# Autodesk Inventor assembly: Assembly2
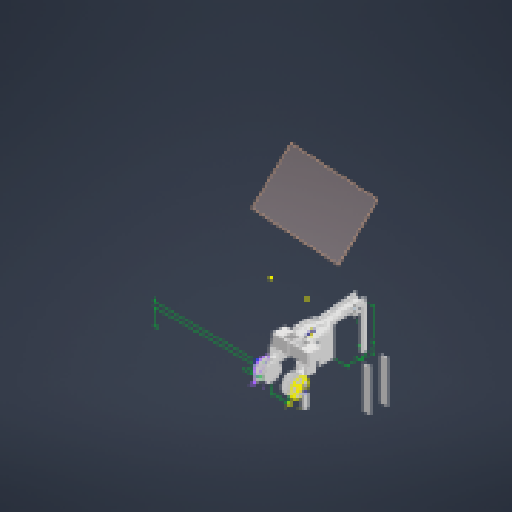
[picture p0: Inventor's stored thumbnail of the model, 512x512]
Saved by Autodesk Inventor 2026.2 (Build 302298000, 298)
## iProperties
Created: 2026-02-23
Part Number: Assembly2
Document SubType Name: Assembly
Designer: danda
Author: danda
## Documents named in this file (17)
- C:\Users\danda\BOM-project\Project\CAD\sorting\Assembly2.iam
- C:\Users\danda\BOM-project\Project\CAD\sorting\Towerpro Micro Servo 9g\Towerpro Micro Servo 9g\Towerpro Micro Servo 9g.ipt
- C:\Users\danda\BOM-project\Project\CAD\sorting\gate2.ipt
- C:\Users\danda\BOM-project\Project\CAD\sorting\wheel.ipt
- C:\Users\danda\BOM-project\Project\CAD\sorting\motorwheelstand.ipt
- C:\Users\danda\BOM-project\Project\CAD\sorting\leftcollection.ipt
- C:\Users\danda\BOM-project\Project\CAD\sorting\rightcollection.ipt
- C:\Users\danda\Downloads\ir-sensor-7.snapshot.2\Assembly2.iam
- C:\Users\danda\BOM-project\Project\CAD\sorting\wheel_MIR.ipt
- C:\Users\danda\BOM-project\Project\CAD\sorting\Towerpro Micro Servo 9g\Towerpro Micro Servo 9g\Towerpro Micro Servo 9g_MIR.ipt
- C:\Users\danda\BOM-project\Project\CAD\sorting\motorwheelstand_MIR.ipt
- C:\Users\danda\BOM-project\Project\CAD\sorting\middleslide\midlleslide.iam
- C:\Users\danda\BOM-project\Project\CAD\sorting\inslide\inslide.iam
- C:\Users\danda\BOM-project\Project\CAD\sorting\Towerpro Micro Servo 9g\Towerpro Micro Servo 9g\Assembly4.iam
- C:\Users\danda\BOM-project\Project\CAD\sorting\outstorage.ipt
- C:\Users\danda\BOM-project\Project\CAD\sorting\protostand.ipt
- C:\Users\danda\BOM-project\Project\CAD\sorting\protostand2.ipt
## Components (19 placed, 16 different names)
1. gate2:1 — Insert:7
2. wheel:1 — Insert:3, Mate:100, Flush:68
3. Towerpro Micro Servo 9g:4 — Mate:61, Mate:62, Mate:63, Insert:3
4. motorwheelstand:1 — Mate:61, Mate:62, Mate:63, Flush:50, Flush:58, Mate:88
5. leftcollection:1 — Flush:41, Flush:57, Mate:83, Mate:85, Mate:98, Flush:64, Flush:67, Flush:68
6. rightcollection:1 — Flush:57, Mate:84, Mate:86, Mate:99, Flush:65, Flush:66
7. Assembly2:1 [sub-assembly] — Mate:92, Mate:93, Mate:94
8. wheel_MIR:1 — Insert:4, Mate:101, Flush:69
9. Towerpro Micro Servo 9g_MIR:1 — Insert:4, Mate:74, Mate:75, Mate:76
10. motorwheelstand_MIR:1 — Mate:74, Mate:75, Mate:76, Flush:50, Flush:58
11. midlleslide:1 [sub-assembly] — Mate:83, Mate:84, Mate:85, Mate:86, Flush:60, Mate:90, Mate:91, Mate:96, Insert:5, Insert:6
12. inslide:1 [sub-assembly] — Flush:60, Mate:90, Mate:91, Mate:92, Mate:93, Mate:94, Mate:102, Mate:103, Mate:104, Mate:105, Mate:106, Mate:107
13. Assembly4:1 [sub-assembly] — Mate:96, Insert:5, Insert:6, Insert:7, Mate:112
14. outstorage:1 — Mate:98, Flush:64, Flush:67, Mate:100
15. outstorage:2 — Mate:99, Flush:65, Flush:66, Mate:101, Flush:69
16. protostand:1 — Mate:102, Mate:104, Mate:106, Mate:110, Mate:113
17. protostand:2 — Mate:103, Mate:105, Mate:107
18. protostand2:1 — Mate:112
19. protostand2:2
## Relationships (46: Mate 30, Flush 11, Insert 5)
- Mate:61: Towerpro Micro Servo 9g:4 ↔ motorwheelstand:1
- Mate:62: Towerpro Micro Servo 9g:4 ↔ motorwheelstand:1
- Mate:63: Towerpro Micro Servo 9g:4 ↔ motorwheelstand:1
- Insert:3: wheel:1 ↔ Towerpro Micro Servo 9g:4
- Flush:41 (2.54 mm): leftcollection:1
- Insert:4: wheel_MIR:1 ↔ Towerpro Micro Servo 9g_MIR:1
- Mate:74: Towerpro Micro Servo 9g_MIR:1 ↔ motorwheelstand_MIR:1
- Mate:75: Towerpro Micro Servo 9g_MIR:1 ↔ motorwheelstand_MIR:1
- Mate:76: Towerpro Micro Servo 9g_MIR:1 ↔ motorwheelstand_MIR:1
- Flush:50: motorwheelstand:1 ↔ motorwheelstand_MIR:1
- Flush:57: leftcollection:1 ↔ rightcollection:1
- Mate:83: leftcollection:1 ↔ midlleslide:1
- Mate:84: rightcollection:1 ↔ midlleslide:1
- Mate:85: leftcollection:1 ↔ midlleslide:1
- Mate:86: rightcollection:1 ↔ midlleslide:1
- Flush:58: motorwheelstand:1 ↔ motorwheelstand_MIR:1
- Mate:88: motorwheelstand:1
- Flush:60: midlleslide:1 ↔ inslide:1
- Mate:90: midlleslide:1 ↔ inslide:1
- Mate:91: midlleslide:1 ↔ inslide:1
- Mate:92: Assembly2:1 ↔ inslide:1
- Mate:93: Assembly2:1 ↔ inslide:1
- Mate:94: Assembly2:1 ↔ inslide:1
- Mate:96: midlleslide:1 ↔ Assembly4:1
- Insert:5: midlleslide:1 ↔ Assembly4:1
- Insert:6: midlleslide:1 ↔ Assembly4:1
- Insert:7: gate2:1 ↔ Assembly4:1
- Mate:98: leftcollection:1 ↔ outstorage:1
- Mate:99: rightcollection:1 ↔ outstorage:2
- Flush:64: leftcollection:1 ↔ outstorage:1
- Flush:65: rightcollection:1 ↔ outstorage:2
- Flush:66: rightcollection:1 ↔ outstorage:2
- Flush:67: leftcollection:1 ↔ outstorage:1
- Mate:100: wheel:1 ↔ outstorage:1
- Mate:101: wheel_MIR:1 ↔ outstorage:2
- Flush:68: wheel:1 ↔ leftcollection:1
- Flush:69: wheel_MIR:1 ↔ outstorage:2
- Mate:102: inslide:1 ↔ protostand:1
- Mate:103: inslide:1 ↔ protostand:2
- Mate:104: inslide:1 ↔ protostand:1
- Mate:105: inslide:1 ↔ protostand:2
- Mate:106: inslide:1 ↔ protostand:1
- Mate:107: inslide:1 ↔ protostand:2
- Mate:110: protostand:1
- Mate:112: Assembly4:1 ↔ protostand2:1
- Mate:113: protostand:1
